# Autodesk Inventor assembly: 상단 조립품
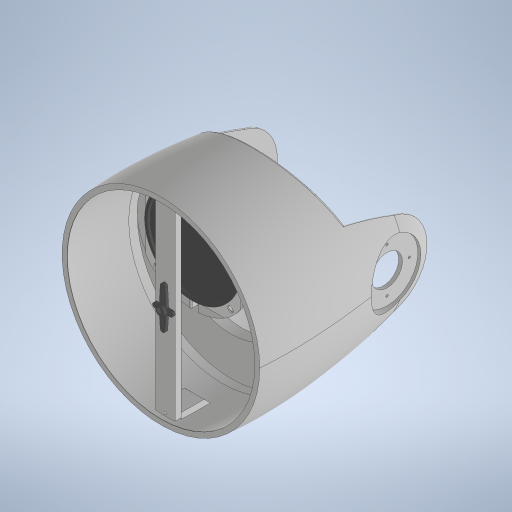
[picture p0: Inventor's stored thumbnail of the model, 512x512]
Saved by Autodesk Inventor 2023.1 (Build 271208000, 208)
## iProperties
Created: 2022-08-14
Part Number: 상단 조립품
Document SubType Name: Assembly
Designer: fly01
Author: fly01
## Documents named in this file (5)
- C:\Users\fly01\Desktop\PAI설계 2\조림품\상단 조립품.iam
- C:\Users\fly01\Desktop\PAI설계 2\범용 부품\스피커.ipt
- C:\Users\fly01\Desktop\PAI설계 2\출력품\body_top.ipt
- C:\Users\fly01\Desktop\PAI설계 2\출력품\상단 서보모터 고정 판.ipt
- C:\Users\fly01\Desktop\PAI설계 2\범용 부품\180도 서보모터 십자축.ipt
## Components (4 placed, 4 different names)
1. 스피커:1 — 삽입:1
2. body_top:1 — 삽입:1, 삽입:4, 삽입:5
3. 상단 서보모터 고정 판:1 — 삽입:2, 삽입:3, 삽입:4, 삽입:5
4. 180도 서보모터 십자축:1 — 삽입:2, 삽입:3
## Relationships (5: Insert 5)
- 삽입:1 [Insert]: 스피커:1 ↔ body_top:1
- 삽입:2 [Insert]: 상단 서보모터 고정 판:1 ↔ 180도 서보모터 십자축:1
- 삽입:3 [Insert]: 상단 서보모터 고정 판:1 ↔ 180도 서보모터 십자축:1
- 삽입:4 [Insert]: body_top:1 ↔ 상단 서보모터 고정 판:1
- 삽입:5 [Insert]: body_top:1 ↔ 상단 서보모터 고정 판:1
